# Autodesk Inventor assembly: frame
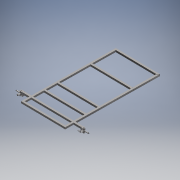
[picture p0: Inventor's stored thumbnail of the model, 180x180]
Saved by Autodesk Inventor 2019 (Build 230136000, 136)
## iProperties
Created: 2019-04-23
Part Number: frame
Document SubType Name: Weldment
Designer: Callum Snowden
Weld Material: Welded Aluminum-6061
Mass: 16255.4 g
Surface Area: 16630.1 cm^2
Volume: 2070.75 cm^3
Density: 7.85 g/cm^3
Author: Callum Snowden
## iProperties of the stored document 59935K730_METRIC BALL JOINT ROD END.ipt
Created: 2012-02-13
Part Number: 59935K730_METRIC BALL JOINT ROD END
Material: Generic
Description: STEP AP203
Document SubType Name: Modeling
Designer: callum.snowden
Density: 1 g/cm^3
Appearance: Default
Title: 59935K73.step
Author: jim
Revision Number: ANY
Sending System: SolidWorks 2009
Preprocessor: SwSTEP 2.0
## Documents named in this file (32)
- C:\Users\callum.snowden\Documents\GitHub\clasohlsonkart\mechanical\frame\frame.iam
- C:\Users\callum.snowden\Documents\GitHub\clasohlsonkart\mechanical\frame\750mm_box_section.ipt
- C:\Users\callum.snowden\Documents\GitHub\clasohlsonkart\mechanical\frame\1500mm_box_section.ipt
- C:\Users\callum.snowden\Documents\GitHub\clasohlsonkart\mechanical\frame\1500mm_box_section_MIR.ipt
- C:\Users\callum.snowden\Documents\GitHub\clasohlsonkart\mechanical\frame\690mm_box_section.ipt
- C:\Users\callum.snowden\Documents\GitHub\clasohlsonkart\mechanical\frame\1250mm_box_section.ipt
- C:\Users\callum.snowden\Documents\GitHub\clasohlsonkart\mechanical\frame\140mm_box_section.ipt
- C:\Users\callum.snowden\Documents\GitHub\clasohlsonkart\mechanical\frame\steering_kingpin_left_assy.iam
- C:\Users\callum.snowden\Documents\GitHub\clasohlsonkart\mechanical\frame\steering_kingpin_right_assy.iam
- **C:\Users\callum.snowden\Documents\GitHub\clasohlsonkart\mechanical\frame\frame.iam*LocalDocs*xZoon433zYuoselos1mkdkxui3c*59935K730_METRIC BALL JOINT ROD END.ipt
- C:\Users\callum.snowden\Documents\Inventor\Content Center Files\R2019\en-US\BS 4168(7)\BS 4168 - 8 x 16.ipt
- C:\Users\callum.snowden\Documents\Inventor\Content Center Files\R2019\en-US\BS 4320(2)\BS 4320 - M8 (Form B).ipt
- C:\Users\callum.snowden\Documents\Inventor\Content Center Files\R2019\en-US\ANSI B18.16.3M(2)\ANSI B18.16.3M - Property Class 5 and 10 - Metric M8 x 1.25 Top Insert Type.ipt
- C:\Users\callum.snowden\Documents\GitHub\clasohlsonkart\mechanical\frame\frame\AIP\FEA\cutzhkwf4.fins
- C:\Users\callum.snowden\Documents\GitHub\clasohlsonkart\mechanical\frame\frame\AIP\FEA\cutzhkwg0.fsat
- C:\Users\callum.snowden\Documents\GitHub\clasohlsonkart\mechanical\frame\frame\AIP\FEA\cutzhkwg0.ftes
- C:\Users\callum.snowden\Documents\GitHub\clasohlsonkart\mechanical\frame\frame\AIP\FEA\cutzhkwg0.fwiz
- C:\Users\callum.snowden\Documents\GitHub\clasohlsonkart\mechanical\frame\frame\AIP\FEA\cutzhkwio.fmsh
- C:\Users\callum.snowden\Documents\GitHub\clasohlsonkart\mechanical\frame\frame\AIP\FEA\cutzhkwip.fres
- C:\Users\callum.snowden\Documents\GitHub\clasohlsonkart\mechanical\frame\frame\AIP\FEA\cuvsryc0w.fins
- C:\Users\callum.snowden\Documents\GitHub\clasohlsonkart\mechanical\frame\frame\AIP\FEA\cuvsryc0w.fsat
- C:\Users\callum.snowden\Documents\GitHub\clasohlsonkart\mechanical\frame\frame\AIP\FEA\cuvsryc0w.ftes
- C:\Users\callum.snowden\Documents\GitHub\clasohlsonkart\mechanical\frame\frame\AIP\FEA\cuvsryc0w.fwiz
- C:\Users\callum.snowden\Documents\GitHub\clasohlsonkart\mechanical\frame\frame\AIP\FEA\cuvsrycbk.fmsh
- C:\Users\callum.snowden\Documents\GitHub\clasohlsonkart\mechanical\frame\frame\AIP\FEA\cuvsrycbl.fres
- C:\Users\callum.snowden\Documents\GitHub\clasohlsonkart\mechanical\frame\59935K730_METRIC BALL JOINT ROD END.STEP
- C:\Users\callum.snowden\Documents\GitHub\clasohlsonkart\mechanical\frame\frame\AIP\FEA\cuwrj3ngg.fins
- C:\Users\callum.snowden\Documents\GitHub\clasohlsonkart\mechanical\frame\frame\AIP\FEA\cuwrj3ngg.fsat
- C:\Users\callum.snowden\Documents\GitHub\clasohlsonkart\mechanical\frame\frame\AIP\FEA\cuwrj3ngg.ftes
- C:\Users\callum.snowden\Documents\GitHub\clasohlsonkart\mechanical\frame\frame\AIP\FEA\cuwrj3ngg.fwiz
- C:\Users\callum.snowden\Documents\GitHub\clasohlsonkart\mechanical\frame\frame\AIP\FEA\cuwrj3ns0.fmsh
- C:\Users\callum.snowden\Documents\GitHub\clasohlsonkart\mechanical\frame\frame\AIP\FEA\cuwrj3ns1.fres
## Components (20 placed, 12 different names)
1. 750mm_box_section:1 — Rigid:11
2. 750mm_box_section:2 — Rigid:3, Rigid:8
3. 1500mm_box_section:1 — Rigid:3, Rigid:4, Rigid:5, Rigid:6
4. 1500mm_box_section_MIR:1 — Rigid:7, Rigid:8
5. 690mm_box_section:1 — Rigid:4
6. 690mm_box_section:2 — Rigid:6
7. 690mm_box_section:3 — Rigid:5
8. 1250mm_box_section:1 — Rigid:7, Rigid:9, Rigid:10, Rigid:12, Rigid:13
9. 140mm_box_section:1 — Rigid:10
10. 140mm_box_section:2 — Rigid:9, Rigid:11
11. steering_kingpin_left_assy:1 [sub-assembly] — Rigid:12, Rotational:2, Rigid:14, Angle:1
12. steering_kingpin_right_assy:1 [sub-assembly] — Rigid:13, Rotational:1, Rotational:5, Angle:2
13. 59935K730_METRIC BALL JOINT ROD END:1 — Rotational:1, Rotational:4, Angle:2
14. 59935K730_METRIC BALL JOINT ROD END:2 — Rotational:2, Rotational:3, Angle:1
15. BS 4168 : Part 7 Hexagon socket screws and wrench keys, metric series- Specification for hexagon socket shoulder screws - Metric 8 x 16:1 — Rotational:3
16. BS 4320 Form AB M8 (Form B):1 — Rigid:14, Rotational:7
17. BS 4320 Form AB M8 (Form B):2 — Rotational:5, Rotational:6
18. BS 4168 : Part 7 Hexagon socket screws and wrench keys, metric series- Specification for hexagon socket shoulder screws - Metric 8 x 16:2 — Rotational:4
19. Prevailing Torque Type Hex Nut - Steel Metric Property Class 5 and 10 - Metric M8 x 1.25 Top Insert Type:1 — Rotational:6
20. Prevailing Torque Type Hex Nut - Steel Metric Property Class 5 and 10 - Metric M8 x 1.25 Top Insert Type:2 — Rotational:7
## Relationships (21: WeldJoint 12, RevoluteJoint 7, Angle 2)
- Rigid:3 [WeldJoint]: 750mm_box_section:2 ↔ 1500mm_box_section:1
- Rigid:4 [WeldJoint]: 1500mm_box_section:1 ↔ 690mm_box_section:1
- Rigid:5 [WeldJoint]: 1500mm_box_section:1 ↔ 690mm_box_section:3
- Rigid:6 [WeldJoint]: 1500mm_box_section:1 ↔ 690mm_box_section:2
- Rigid:7 [WeldJoint]: 1500mm_box_section_MIR:1 ↔ 1250mm_box_section:1
- Rigid:8 [WeldJoint]: 750mm_box_section:2 ↔ 1500mm_box_section_MIR:1
- Rigid:9 [WeldJoint]: 1250mm_box_section:1 ↔ 140mm_box_section:2
- Rigid:10 [WeldJoint]: 1250mm_box_section:1 ↔ 140mm_box_section:1
- Rigid:11 [WeldJoint]: 750mm_box_section:1 ↔ 140mm_box_section:2
- Rigid:12 [WeldJoint]: 1250mm_box_section:1 ↔ steering_kingpin_left_assy:1
- Rigid:13 [WeldJoint]: 1250mm_box_section:1 ↔ steering_kingpin_right_assy:1
- Rotational:1 [RevoluteJoint]: steering_kingpin_right_assy:1 ↔ 59935K730_METRIC BALL JOINT ROD END:1
- Rotational:2 [RevoluteJoint]: steering_kingpin_left_assy:1 ↔ 59935K730_METRIC BALL JOINT ROD END:2
- Rotational:3 [RevoluteJoint]: 59935K730_METRIC BALL JOINT ROD END:2 ↔ BS 4168 : Part 7 Hexagon socket screws and wrench keys, metric series- Specification for hexagon socket shoulder screws - Metric 8 x 16:1
- Rigid:14 [WeldJoint]: steering_kingpin_left_assy:1 ↔ BS 4320 Form AB M8 (Form B):1
- Rotational:4 [RevoluteJoint]: 59935K730_METRIC BALL JOINT ROD END:1 ↔ BS 4168 : Part 7 Hexagon socket screws and wrench keys, metric series- Specification for hexagon socket shoulder screws - Metric 8 x 16:2
- Rotational:5 [RevoluteJoint]: steering_kingpin_right_assy:1 ↔ BS 4320 Form AB M8 (Form B):2
- Rotational:6 [RevoluteJoint]: BS 4320 Form AB M8 (Form B):2 ↔ Prevailing Torque Type Hex Nut - Steel Metric Property Class 5 and 10 - Metric M8 x 1.25 Top Insert Type:1
- Rotational:7 [RevoluteJoint]: BS 4320 Form AB M8 (Form B):1 ↔ Prevailing Torque Type Hex Nut - Steel Metric Property Class 5 and 10 - Metric M8 x 1.25 Top Insert Type:2
- Angle:1 (180 deg): steering_kingpin_left_assy:1 ↔ 59935K730_METRIC BALL JOINT ROD END:2
- Angle:2 (180 deg): steering_kingpin_right_assy:1 ↔ 59935K730_METRIC BALL JOINT ROD END:1
## Named parameters: sa_0 = 0, sa_1 = 0, sa_2 = -100000, sa_3 = -6e-12, sa_4 = -2.6e-12, sa_5 = -79000, sa_6 = 40000
note: some values were not read from the file. Shown as the stored number, unit unknown: "sa_0", "sa_1", "sa_2", "sa_3", "sa_4", "sa_5", "sa_6".
